# Autodesk Inventor assembly: тески1
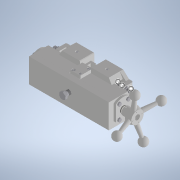
[picture p0: Inventor's stored thumbnail of the model, 180x180]
Saved by Autodesk Inventor 2022 (Build 260153000, 153)
## iProperties
Created: 2021-12-04
Part Number: тески1
Document SubType Name: Assembly
Designer: Украинцев
Author: Украинцев
## Documents named in this file (22)
- D:\Desk\тески\тески1.iam
- D:\Desk\тески\Угольник-10.ipt
- D:\Desk\тески\Губка-2.ipt
- D:\Desk\тески\Призма-5.ipt
- D:\Desk\тески\Крышка-6.ipt
- D:\Desk\тески\Колонка-1.ipt
- D:\Desk\тески\сборка1\Сборка2.iam
- D:\Desk\тески\Фиксатор-11.ipt
- D:\Desk\тески\Втулка-12.ipt
- D:\Desk\тески\Втулка-4.ipt
- D:\Desk\тески\Ручка-09.ipt
- D:\Desk\тески\Рукоятка-8.ipt
- D:\Desk\тески\Гайка-7.ipt
- D:\Desk\тески\болт\Штифт 2.3x20 ГОСТ 3128-70.ipt
- D:\Desk\тески\болт\Болт M8-6gx20 ГОСТ 7808-70.ipt
- D:\Desk\тески\болт\Винт M10-6gx40 ГОСТ 1482-84.ipt
- D:\Desk\тески\болт\Гайка M10-6H ГОСТ 5916-70.ipt
- D:\Desk\тески\болт\Винт M8-6gx12 ГОСТ 1491-80.ipt
- D:\Desk\тески\болт\Штифт 2.8x30 ГОСТ 3128-70.ipt
- D:\Desk\тески\болт\Винт M8-6gx25 ГОСТ 1477-93.ipt
- D:\Desk\тески\болт\Болт M10-6gx30 ГОСТ 7808-70.ipt
- D:\Desk\тески\болт\Болт M16-6gx45 ГОСТ 7808-70.ipt
## Components (58 placed, 21 different names)
1. Угольник-10:1 — Совмещение:1, Заподлицо:1, Совмещение:2, Совмещение:3, Заподлицо:2, Совмещение:4, Совмещение:39, Совмещение:43, Совмещение:46, Совмещение:59, Совмещение:60, Совмещение:61, Совмещение:62
2. Губка-2:1 — Совмещение:3, Заподлицо:2, Совмещение:4, Совмещение:5, Совмещение:6, Совмещение:11, Совмещение:16, Заподлицо:5, Заподлицо:6, Совмещение:20, Совмещение:40, Совмещение:55, Заподлицо:9, Совмещение:57, Заподлицо:11
3. Губка-2:2 — Совмещение:1, Заподлицо:1, Совмещение:2, Совмещение:7, Совмещение:8, Совмещение:9, Совмещение:10, Совмещение:15, Заподлицо:3, Заподлицо:4, Совмещение:18, Совмещение:41, Совмещение:56, Заподлицо:10, Совмещение:58, Заподлицо:12
4. Призма-5:1 — Совмещение:7, Совмещение:8, Совмещение:64
5. Призма-5:2 — Совмещение:5, Совмещение:6, Совмещение:63
6. Крышка-6:1 — Совмещение:16, Заподлицо:5, Заподлицо:6, Совмещение:38, Совмещение:47, Совмещение:48, Совмещение:49
7. Крышка-6:2 — Совмещение:15, Заподлицо:3, Заподлицо:4, Совмещение:34, Совмещение:35, Совмещение:44, Совмещение:45
8. Колонка-1:1 — Совмещение:9, Совмещение:10, Совмещение:14, Совмещение:42, Совмещение:43
9. Сборка2:1 [sub-assembly] — Совмещение:11, Совмещение:12, Совмещение:13, Совмещение:17, Совмещение:19, Совмещение:25, Совмещение:26
10. Фиксатор-11:1 — Совмещение:12, Совмещение:13, Совмещение:14, Совмещение:42, Совмещение:50, Совмещение:51, Совмещение:52, Совмещение:53, Совмещение:54, Заподлицо:8
11. Втулка-12:1 — Совмещение:17, Совмещение:18, Совмещение:28, Совмещение:29
12. Втулка-4:1 — Совмещение:19, Совмещение:20, Совмещение:30, Совмещение:31
13. Гайка-7:1 — Совмещение:23, Совмещение:24, Совмещение:25, Совмещение:26, Совмещение:27, Заподлицо:7
14. Винт ГОСТ 1491-80 M 8 x 12:9 — Совмещение:50, Совмещение:51
15. Винт ГОСТ 1491-80 M 8 x 12:10 — Совмещение:52, Совмещение:53
16. Штифты 2 ГОСТ 3128-70 8 x  30:1 — Совмещение:54, Заподлицо:8
17. Винт ГОСТ 1477-93 M8x25-B:1 — Совмещение:55, Заподлицо:9
18. Винт ГОСТ 1477-93 M8x25-B:2 — Совмещение:56, Заподлицо:10
19. Винт ГОСТ 1477-93 M8x25-B:3 — Совмещение:57, Заподлицо:11
20. Винт ГОСТ 1477-93 M8x25-B:4 — Совмещение:58, Заподлицо:12
21. Болт ГОСТ 7808-70 M10-6gx30:1 — Совмещение:59, Совмещение:60
22. Болт ГОСТ 7808-70 M16-6gx45:1 — Совмещение:61, Совмещение:62
23. Штифты 2 ГОСТ 3128-70 3 x  20:1 — Совмещение:27, Заподлицо:7
24. Штифты 2 ГОСТ 3128-70 3 x  20:2
25. Штифты 2 ГОСТ 3128-70 3 x  20:3
26. Штифты 2 ГОСТ 3128-70 3 x  20:4
27. Болт ГОСТ 7808-70 M8-6gx20:1 — Совмещение:28, Совмещение:29, Совмещение:41
28. Болт ГОСТ 7808-70 M8-6gx20:2
29. Болт ГОСТ 7808-70 M8-6gx20:3
30. Болт ГОСТ 7808-70 M8-6gx20:4
31. Болт ГОСТ 7808-70 M8-6gx20:5 — Совмещение:30, Совмещение:31, Совмещение:40
32. Болт ГОСТ 7808-70 M8-6gx20:6
33. Болт ГОСТ 7808-70 M8-6gx20:7
34. Болт ГОСТ 7808-70 M8-6gx20:8
35. Гайка ГОСТ 5916-70 M10:1 — Совмещение:32, Совмещение:33, Совмещение:35
36. Винт ГОСТ 1482-84 M 10 x 40:1 — Совмещение:32, Совмещение:33, Совмещение:34
37. Гайка ГОСТ 5916-70 M10:2
38. Винт ГОСТ 1482-84 M 10 x 40:2 — Совмещение:64
39. Винт ГОСТ 1482-84 M 10 x 40:3 — Совмещение:36, Совмещение:37, Совмещение:38
40. Гайка ГОСТ 5916-70 M10:3 — Совмещение:36, Совмещение:37, Совмещение:49
41. Винт ГОСТ 1482-84 M 10 x 40:4 — Совмещение:63
42. Гайка ГОСТ 5916-70 M10:4
43. Рукоятка-8:1 — Совмещение:21, Совмещение:22, Совмещение:23, Совмещение:24
44. Ручка-09:1 — Совмещение:21, Совмещение:22
45. Рукоятка-8:2
46. Ручка-09:2
47. Рукоятка-8:3
48. Ручка-09:3
49. Рукоятка-8:4
50. Ручка-09:4
51. Винт ГОСТ 1491-80 M 8 x 12:1 — Совмещение:44, Совмещение:45
52. Винт ГОСТ 1491-80 M 8 x 12:2
53. Винт ГОСТ 1491-80 M 8 x 12:3
54. Винт ГОСТ 1491-80 M 8 x 12:4
55. Винт ГОСТ 1491-80 M 8 x 12:5 — Совмещение:47, Совмещение:48
56. Винт ГОСТ 1491-80 M 8 x 12:6
57. Винт ГОСТ 1491-80 M 8 x 12:7
58. Винт ГОСТ 1491-80 M 8 x 12:8
## Component patterns: (4 elements, first: Штифты 2 ГОСТ 3128-70 3 x  20:1), (4 elements, first: Болт ГОСТ 7808-70 M8-6gx20:1), (4 elements, first: Болт ГОСТ 7808-70 M8-6gx20:5), (2 elements, first: Гайка ГОСТ 5916-70 M10:1 + Винт ГОСТ 1482-84 M 10 x 40:1), (2 elements, first: Винт ГОСТ 1482-84 M 10 x 40:3 + Гайка ГОСТ 5916-70 M10:3), (4 elements, first: Рукоятка-8:1 + Ручка-09:1), (4 elements, first: Винт ГОСТ 1491-80 M 8 x 12:1), (4 elements, first: Винт ГОСТ 1491-80 M 8 x 12:5)
## Relationships (76: Mate 64, Flush 12)
- Совмещение:1 [Mate]: Угольник-10:1 ↔ Губка-2:2
- Заподлицо:1 [Flush]: Угольник-10:1 ↔ Губка-2:2
- Совмещение:2 [Mate]: Угольник-10:1 ↔ Губка-2:2
- Совмещение:3 [Mate]: Угольник-10:1 ↔ Губка-2:1
- Заподлицо:2 [Flush]: Угольник-10:1 ↔ Губка-2:1
- Совмещение:4 [Mate]: Угольник-10:1 ↔ Губка-2:1
- Совмещение:5 [Mate]: Губка-2:1 ↔ Призма-5:2
- Совмещение:6 [Mate]: Губка-2:1 ↔ Призма-5:2
- Совмещение:7 [Mate]: Губка-2:2 ↔ Призма-5:1
- Совмещение:8 [Mate]: Губка-2:2 ↔ Призма-5:1
- Совмещение:9 [Mate]: Губка-2:2 ↔ Колонка-1:1
- Совмещение:10 [Mate] (1 mm): Губка-2:2 ↔ Колонка-1:1
- Совмещение:11 [Mate]: Губка-2:1 ↔ Сборка2:1
- Совмещение:12 [Mate]: Сборка2:1 ↔ Фиксатор-11:1
- Совмещение:13 [Mate]: Сборка2:1 ↔ Фиксатор-11:1
- Совмещение:14 [Mate]: Колонка-1:1 ↔ Фиксатор-11:1
- Совмещение:15 [Mate]: Губка-2:2 ↔ Крышка-6:2
- Заподлицо:3 [Flush]: Губка-2:2 ↔ Крышка-6:2
- Заподлицо:4 [Flush]: Губка-2:2 ↔ Крышка-6:2
- Совмещение:16 [Mate]: Губка-2:1 ↔ Крышка-6:1
- Заподлицо:5 [Flush]: Губка-2:1 ↔ Крышка-6:1
- Заподлицо:6 [Flush]: Губка-2:1 ↔ Крышка-6:1
- Совмещение:17 [Mate]: Сборка2:1 ↔ Втулка-12:1
- Совмещение:18 [Mate]: Губка-2:2 ↔ Втулка-12:1
- Совмещение:19 [Mate]: Сборка2:1 ↔ Втулка-4:1
- Совмещение:20 [Mate]: Губка-2:1 ↔ Втулка-4:1
- Совмещение:21 [Mate]: Рукоятка-8:1 ↔ Ручка-09:1
- Совмещение:22 [Mate]: Рукоятка-8:1 ↔ Ручка-09:1
- Совмещение:23 [Mate]: Гайка-7:1 ↔ Рукоятка-8:1
- Совмещение:24 [Mate]: Гайка-7:1 ↔ Рукоятка-8:1
- Совмещение:25 [Mate]: Сборка2:1 ↔ Гайка-7:1
- Совмещение:26 [Mate]: Сборка2:1 ↔ Гайка-7:1
- Совмещение:27 [Mate]: Гайка-7:1 ↔ Штифты 2 ГОСТ 3128-70 3 x  20:1
- Заподлицо:7 [Flush] (1 mm): Гайка-7:1 ↔ Штифты 2 ГОСТ 3128-70 3 x  20:1
- Совмещение:28 [Mate]: Втулка-12:1 ↔ Болт ГОСТ 7808-70 M8-6gx20:1
- Совмещение:29 [Mate]: Втулка-12:1 ↔ Болт ГОСТ 7808-70 M8-6gx20:1
- Совмещение:30 [Mate]: Втулка-4:1 ↔ Болт ГОСТ 7808-70 M8-6gx20:5
- Совмещение:31 [Mate]: Втулка-4:1 ↔ Болт ГОСТ 7808-70 M8-6gx20:5
- Совмещение:32 [Mate]: Гайка ГОСТ 5916-70 M10:1 ↔ Винт ГОСТ 1482-84 M 10 x 40:1
- Совмещение:33 [Mate] (3.5 mm): Гайка ГОСТ 5916-70 M10:1 ↔ Винт ГОСТ 1482-84 M 10 x 40:1
- Совмещение:34 [Mate]: Крышка-6:2 ↔ Винт ГОСТ 1482-84 M 10 x 40:1
- Совмещение:35 [Mate]: Крышка-6:2 ↔ Гайка ГОСТ 5916-70 M10:1
- Совмещение:36 [Mate]: Винт ГОСТ 1482-84 M 10 x 40:3 ↔ Гайка ГОСТ 5916-70 M10:3
- Совмещение:37 [Mate] (3.5 mm): Винт ГОСТ 1482-84 M 10 x 40:3 ↔ Гайка ГОСТ 5916-70 M10:3
- Совмещение:38 [Mate]: Крышка-6:1 ↔ Винт ГОСТ 1482-84 M 10 x 40:3
- Совмещение:39 [Mate]: Угольник-10:1
- Совмещение:40 [Mate]: Губка-2:1 ↔ Болт ГОСТ 7808-70 M8-6gx20:5
- Совмещение:41 [Mate]: Губка-2:2 ↔ Болт ГОСТ 7808-70 M8-6gx20:1
- Совмещение:42 [Mate]: Колонка-1:1 ↔ Фиксатор-11:1
- Совмещение:43 [Mate]: Угольник-10:1 ↔ Колонка-1:1
- Совмещение:44 [Mate]: Крышка-6:2 ↔ Винт ГОСТ 1491-80 M 8 x 12:1
- Совмещение:45 [Mate]: Крышка-6:2 ↔ Винт ГОСТ 1491-80 M 8 x 12:1
- Совмещение:46 [Mate]: Угольник-10:1
- Совмещение:47 [Mate]: Крышка-6:1 ↔ Винт ГОСТ 1491-80 M 8 x 12:5
- Совмещение:48 [Mate]: Крышка-6:1 ↔ Винт ГОСТ 1491-80 M 8 x 12:5
- Совмещение:49 [Mate]: Крышка-6:1 ↔ Гайка ГОСТ 5916-70 M10:3
- Совмещение:50 [Mate]: Фиксатор-11:1 ↔ Винт ГОСТ 1491-80 M 8 x 12:9
- Совмещение:51 [Mate]: Фиксатор-11:1 ↔ Винт ГОСТ 1491-80 M 8 x 12:9
- Совмещение:52 [Mate]: Фиксатор-11:1 ↔ Винт ГОСТ 1491-80 M 8 x 12:10
- Совмещение:53 [Mate]: Фиксатор-11:1 ↔ Винт ГОСТ 1491-80 M 8 x 12:10
- Совмещение:54 [Mate]: Фиксатор-11:1 ↔ Штифты 2 ГОСТ 3128-70 8 x  30:1
- Заподлицо:8 [Flush]: Фиксатор-11:1 ↔ Штифты 2 ГОСТ 3128-70 8 x  30:1
- Совмещение:55 [Mate]: Губка-2:1 ↔ Винт ГОСТ 1477-93 M8x25-B:1
- Заподлицо:9 [Flush]: Губка-2:1 ↔ Винт ГОСТ 1477-93 M8x25-B:1
- Совмещение:56 [Mate]: Губка-2:2 ↔ Винт ГОСТ 1477-93 M8x25-B:2
- Заподлицо:10 [Flush]: Губка-2:2 ↔ Винт ГОСТ 1477-93 M8x25-B:2
- Совмещение:57 [Mate]: Губка-2:1 ↔ Винт ГОСТ 1477-93 M8x25-B:3
- Заподлицо:11 [Flush]: Губка-2:1 ↔ Винт ГОСТ 1477-93 M8x25-B:3
- Совмещение:58 [Mate]: Губка-2:2 ↔ Винт ГОСТ 1477-93 M8x25-B:4
- Заподлицо:12 [Flush]: Губка-2:2 ↔ Винт ГОСТ 1477-93 M8x25-B:4
- Совмещение:59 [Mate]: Угольник-10:1 ↔ Болт ГОСТ 7808-70 M10-6gx30:1
- Совмещение:60 [Mate]: Угольник-10:1 ↔ Болт ГОСТ 7808-70 M10-6gx30:1
- Совмещение:61 [Mate]: Угольник-10:1 ↔ Болт ГОСТ 7808-70 M16-6gx45:1
- Совмещение:62 [Mate] (15 mm): Угольник-10:1 ↔ Болт ГОСТ 7808-70 M16-6gx45:1
- Совмещение:63 [Mate]: Призма-5:2 ↔ Винт ГОСТ 1482-84 M 10 x 40:4
- Совмещение:64 [Mate]: Призма-5:1 ↔ Винт ГОСТ 1482-84 M 10 x 40:2
